# Autodesk Inventor assembly: 4ax_plate_joint_asm
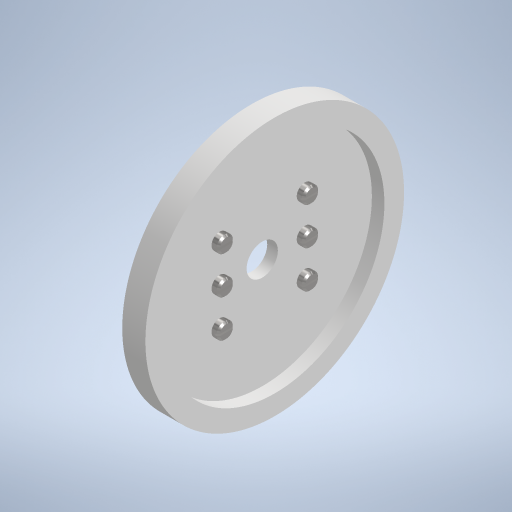
[picture p0: Inventor's stored thumbnail of the model, 512x512]
Saved by Autodesk Inventor 2024 (Build 280153000, 153)
## iProperties
Created: 2025-12-20
Part Number: 4ax_plate_joint_asm
Document SubType Name: Assembly
Designer: schar
Author: schar
## Documents named in this file (3)
- C:\Users\schar\Desktop\projectBlueprint\AMSTS\hardware\4ax_plate_joint_asm.iam
- C:\Users\schar\Desktop\projectBlueprint\AMSTS\hardware\4ax_plate_joint.ipt
- C:\Users\schar\Documents\Inventor\Content Center Files\R2024\en-US\DIN 920\DIN 920 - M5 x 10.ipt
## Components (7 placed, 2 different names)
1. 4ax_plate_joint:1 — Mate:1, Mate:2, Mate:3, Mate:4, Mate:5, Mate:6, Mate:7, Mate:8, Mate:9, Mate:10, Mate:11, Mate:12
2. DIN 920 M5 x 10:1 — Mate:4, Mate:9
3. DIN 920 M5 x 10:2 — Mate:5, Mate:8
4. DIN 920 M5 x 10:3 — Mate:6, Mate:7
5. DIN 920 M5 x 10:4 — Mate:3, Mate:12
6. DIN 920 M5 x 10:5 — Mate:2, Mate:11
7. DIN 920 M5 x 10:6 — Mate:1, Mate:10
## Relationships (12: Mate 12)
- Mate:1: 4ax_plate_joint:1 ↔ DIN 920 M5 x 10:6
- Mate:2: 4ax_plate_joint:1 ↔ DIN 920 M5 x 10:5
- Mate:3: 4ax_plate_joint:1 ↔ DIN 920 M5 x 10:4
- Mate:4: 4ax_plate_joint:1 ↔ DIN 920 M5 x 10:1
- Mate:5: 4ax_plate_joint:1 ↔ DIN 920 M5 x 10:2
- Mate:6: 4ax_plate_joint:1 ↔ DIN 920 M5 x 10:3
- Mate:7: 4ax_plate_joint:1 ↔ DIN 920 M5 x 10:3
- Mate:8: 4ax_plate_joint:1 ↔ DIN 920 M5 x 10:2
- Mate:9: 4ax_plate_joint:1 ↔ DIN 920 M5 x 10:1
- Mate:10: 4ax_plate_joint:1 ↔ DIN 920 M5 x 10:6
- Mate:11: 4ax_plate_joint:1 ↔ DIN 920 M5 x 10:5
- Mate:12: 4ax_plate_joint:1 ↔ DIN 920 M5 x 10:4
